# Autodesk Inventor assembly: Horn
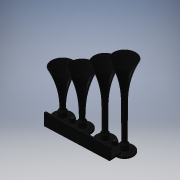
[picture p0: Inventor's stored thumbnail of the model, 180x180]
Saved by Autodesk Inventor 2016 (Build 200138000, 138)
## iProperties
Created: 2016-05-21
Part Number: Horn
Document SubType Name: Assembly
Designer: agmle
Mass: 5016.74 g
Surface Area: 3407.73 cm^2
Volume: 639.076 cm^3
Density: 7.85 g/cm^3
Author: agmle
## Documents named in this file (7)
- C:\Users\agmle\BitTorrent Sync\private\projects\Creekfleet_Timer\hardware\CAD\Remote\Horn.iam
- C:\Users\agmle\BitTorrent Sync\private\projects\Creekfleet_Timer\hardware\CAD\Remote\Diaphragm.ipt
- C:\Users\agmle\BitTorrent Sync\private\projects\Creekfleet_Timer\hardware\CAD\Remote\Horn_A.ipt
- C:\Users\agmle\BitTorrent Sync\private\projects\Creekfleet_Timer\hardware\CAD\Remote\Horn_B.ipt
- C:\Users\agmle\BitTorrent Sync\private\projects\Creekfleet_Timer\hardware\CAD\Remote\Horn_C.ipt
- C:\Users\agmle\BitTorrent Sync\private\projects\Creekfleet_Timer\hardware\CAD\Remote\Horn_D.ipt
- C:\Users\agmle\BitTorrent Sync\private\projects\Creekfleet_Timer\hardware\CAD\Remote\Horn_Bracket.ipt
## Components (7 placed, 6 different names)
1. Diaphragm:1 — Insert:3, Insert:4, Insert:6, Mate:1
2. Diaphragm:2 — Insert:1, Insert:2, Insert:5, Mate:2
3. Horn_A:1 — Insert:1
4. Horn_B:1 — Insert:2
5. Horn_C:1 — Insert:3
6. Horn_D:1 — Insert:4
7. Horn_Bracket:1 — Insert:5, Insert:6, Mate:1, Mate:2
## Relationships (8: Insert 6, Mate 2)
- Insert:1: Diaphragm:2 ↔ Horn_A:1
- Insert:2: Diaphragm:2 ↔ Horn_B:1
- Insert:3: Diaphragm:1 ↔ Horn_C:1
- Insert:4: Diaphragm:1 ↔ Horn_D:1
- Insert:5: Diaphragm:2 ↔ Horn_Bracket:1
- Insert:6: Diaphragm:1 ↔ Horn_Bracket:1
- Mate:1: Diaphragm:1 ↔ Horn_Bracket:1
- Mate:2: Diaphragm:2 ↔ Horn_Bracket:1
